# Autodesk Inventor assembly: J005649
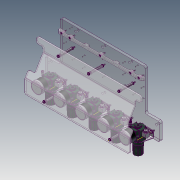
[picture p0: Inventor's stored thumbnail of the model, 180x180]
Saved by Autodesk Inventor 2015 SP1 (Build 190203100, 203)
## iProperties
Created: 2015-05-14
Vendor: HHMI: JRC - ID&F
Document SubType Name: Assembly
Designer: ARNOLDJ
Part Number: J005649
Description: REGULATOR PLATE ASSEMBLY
RuleStatus: InUse
AfterDocSave0: file://Part Number Cleaner
DESIGN DEPARTMENT: HHMI: JRC - ID&F
ALTERED ITEM PART NUMBER: N/A
ALTERED ITEM VENDOR: N/A
ALTERED ITEM DESCRIPTION: N/A
Revision Number: 0
## Documents named in this file (12)
- C:\_WORKSPACE\DATA\COLLABORATION\SVOBODA LAB\MOUSE POSITIONING SYSTEMS\MCAD\BALL SETUP\MBS REG PLATE ASSY.iam
- C:\_WORKSPACE\DATA\COLLABORATION\SVOBODA LAB\MOUSE POSITIONING SYSTEMS\MCAD\BALL SETUP\MBS REG BASE PLATE.ipt
- C:\_WORKSPACE\DATA\COLLABORATION\SVOBODA LAB\MOUSE POSITIONING SYSTEMS\MCAD\BALL SETUP\MBS REGULATOR ASSY.iam
- C:\_WORKSPACE\DATA\COLLABORATION\SVOBODA LAB\MOUSE POSITIONING SYSTEMS\MCAD\BALL SETUP\95947A074.ipt
- C:\_WORKSPACE\DATA\COLLABORATION\SVOBODA LAB\MOUSE POSITIONING SYSTEMS\MCAD\BALL SETUP\93475A230.ipt
- C:\_WORKSPACE\DATA\COLLABORATION\SVOBODA LAB\MOUSE POSITIONING SYSTEMS\MCAD\BALL SETUP\MBS DEFLECTOR SHIELD .ipt
- C:\_WORKSPACE\DATA\COLLABORATION\SVOBODA LAB\MOUSE POSITIONING SYSTEMS\MCAD\BALL SETUP\MBS TROUGH RAIL.ipt
- C:\_WORKSPACE\DATA\COLLABORATION\SVOBODA LAB\MOUSE POSITIONING SYSTEMS\MCAD\BALL SETUP\92010A226.ipt
- C:\_WORKSPACE\DATA\COLLABORATION\SVOBODA LAB\MOUSE POSITIONING SYSTEMS\MCAD\BALL SETUP\92029A152.ipt
- C:\_WORKSPACE\DATA\COLLABORATION\SVOBODA LAB\MOUSE POSITIONING SYSTEMS\MCAD\BALL SETUP\90116A207.ipt
- C:\_WORKSPACE\DATA\COLLABORATION\SVOBODA LAB\MOUSE POSITIONING SYSTEMS\MCAD\BALL SETUP\93475A240.ipt
- C:\_WORKSPACE\DATA\COLLABORATION\SVOBODA LAB\MOUSE POSITIONING SYSTEMS\MCAD\BALL SETUP\92000A320.ipt
## Components (67 placed, 11 different names)
1. MBS REG BASE PLATE:1 — Mate:1, Mate:2, Mate:3, Mate:4, Mate:5, Mate:6, Mate:7, Mate:8, Mate:9, Mate:10, Mate:11, Mate:16, Mate:17, Mate:18, Mate:22, Mate:23, Mate:24, Mate:25, Mate:30, Mate:31, Mate:32, Mate:33, Mate:40, Mate:41, Mate:42, Flush:6, Mate:48, Flush:7, Mate:49, Flush:8, Mate:50, Flush:9, Mate:51, Flush:10, Mate:52
2. 95947A074:1 — Mate:10, Mate:11, Mate:12, Mate:13, Mate:55
3. 95947A074:2 — Mate:12, Mate:13, Mate:19, Mate:20, Mate:21, Mate:54
4. 95947A074:3 — Mate:34, Mate:35, Mate:36, Mate:37, Mate:39
5. 95947A074:4 — Mate:30, Mate:31, Mate:34, Mate:35, Flush:11, Mate:53
6. 95947A074:5 — Mate:4, Mate:5, Mate:28, Mate:29
7. 95947A074:6 — Mate:6, Mate:9, Mate:26, Mate:27
8. 95947A074:7 — Mate:7, Mate:8, Mate:14, Mate:15
9. 93475A230:1 — Mate:14, Mate:15, Mate:65
10. 93475A230:2 — Mate:16, Mate:17
11. 93475A230:3 — Mate:18, Mate:19
12. 93475A230:4 — Mate:28, Mate:29, Mate:63
13. 93475A230:5 — Mate:26, Mate:27, Mate:64
14. 93475A230:6 — Mate:22, Mate:23
15. 93475A230:7 — Mate:24, Mate:25
16. 93475A230:8 — Mate:32, Mate:33
17. 93475A230:9 — Mate:36, Mate:37
18. 93475A230:10 — Mate:20, Mate:21, Mate:38
19. MBS DEFLECTOR SHIELD :1 — Mate:38, Mate:39, Angle:1, Mate:56, Mate:57, Mate:58, Mate:59, Mate:60, Mate:61, Mate:62
20. MBS TROUGH RAIL:1 — Mate:40, Mate:41, Mate:42, Mate:43, Flush:1, Mate:44, Mate:45, Mate:46, Mate:47, Flush:2, Flush:3, Flush:4, Flush:5
21. 92010A226:1 — Mate:43, Flush:1
22. 92010A226:2 — Mate:45, Flush:5
23. 92010A226:3 — Mate:44, Flush:4
24. 92010A226:4 — Mate:46, Flush:3
25. 92010A226:5 — Mate:47, Flush:2
26. 92029A152:1 — Flush:6, Mate:48
27. 92029A152:2 — Flush:7, Mate:49
28. 92029A152:3 — Flush:8, Mate:50
29. 92029A152:4 — Flush:11, Mate:53
30. 92029A152:5 — Mate:54, Mate:55
31. 92029A152:6 — Flush:10, Mate:52
32. 92029A152:9 — Flush:9, Mate:51
33. 93475A230:11 — Mate:57, Mate:63, Mate:70, Mate:71
34. 93475A230:12 — Mate:56, Mate:64, Mate:68, Mate:69
35. 93475A230:13 — Mate:59, Mate:61, Mate:72, Mate:73
36. 93475A230:14 — Mate:58, Mate:65, Mate:66, Mate:67
37. 93475A230:15 — Mate:60, Mate:62, Mate:74, Mate:75
38. 90116A207:1 — Mate:74, Mate:75
39. 90116A207:2 — Mate:72, Mate:73
40. 90116A207:3 — Mate:70, Mate:71
41. 90116A207:4 — Mate:66, Mate:67
42. 90116A207:5 — Mate:68, Mate:69
43. MBS REGULATOR ASSY:1 [sub-assembly] — Mate:1, Mate:2, Mate:3, Mate:76, Mate:77, Mate:78, Mate:79
44. MBS REGULATOR ASSY:2 [sub-assembly]
45. MBS REGULATOR ASSY:3 [sub-assembly]
46. MBS REGULATOR ASSY:4 [sub-assembly]
47. MBS REGULATOR ASSY:5 [sub-assembly]
48. 93475A240:2 — Mate:78, Mate:79, Mate:82, Mate:83
49. 92000A320:2 — Mate:82, Mate:83
50. 93475A240:1 — Mate:76, Mate:77, Mate:80, Mate:81
51. 92000A320:1 — Mate:80, Mate:81
52. 93475A240:3
53. 92000A320:3
54. 93475A240:4
55. 92000A320:4
56. 93475A240:5
57. 92000A320:5
58. 93475A240:6
59. 92000A320:6
60. 93475A240:7
61. 92000A320:7
62. 93475A240:8
63. 92000A320:8
64. 93475A240:9
65. 92000A320:9
66. 93475A240:10
67. 92000A320:10
## Component patterns: (5 elements, first: MBS REGULATOR ASSY:1), (5 elements, first: 93475A240:2 + 92000A320:2 + 93475A240:1 + 92000A320:1)
## Relationships (95: Mate 83, Flush 11, Angle 1)
- Mate:1: MBS REG BASE PLATE:1 ↔ MBS REGULATOR ASSY:1
- Mate:2: MBS REG BASE PLATE:1 ↔ MBS REGULATOR ASSY:1
- Mate:3: MBS REG BASE PLATE:1 ↔ MBS REGULATOR ASSY:1
- Mate:4: MBS REG BASE PLATE:1 ↔ 95947A074:5
- Mate:5 (0.889 mm): MBS REG BASE PLATE:1 ↔ 95947A074:5
- Mate:6: MBS REG BASE PLATE:1 ↔ 95947A074:6
- Mate:7: MBS REG BASE PLATE:1 ↔ 95947A074:7
- Mate:8 (0.889 mm): MBS REG BASE PLATE:1 ↔ 95947A074:7
- Mate:9 (0.889 mm): MBS REG BASE PLATE:1 ↔ 95947A074:6
- Mate:10: MBS REG BASE PLATE:1 ↔ 95947A074:1
- Mate:11 (0.889 mm): MBS REG BASE PLATE:1 ↔ 95947A074:1
- Mate:12: 95947A074:1 ↔ 95947A074:2
- Mate:13: 95947A074:1 ↔ 95947A074:2
- Mate:14: 95947A074:7 ↔ 93475A230:1
- Mate:15: 95947A074:7 ↔ 93475A230:1
- Mate:16: MBS REG BASE PLATE:1 ↔ 93475A230:2
- Mate:17: MBS REG BASE PLATE:1 ↔ 93475A230:2
- Mate:18: MBS REG BASE PLATE:1 ↔ 93475A230:3
- Mate:19: 95947A074:2 ↔ 93475A230:3
- Mate:20: 95947A074:2 ↔ 93475A230:10
- Mate:21: 95947A074:2 ↔ 93475A230:10
- Mate:22: MBS REG BASE PLATE:1 ↔ 93475A230:6
- Mate:23: MBS REG BASE PLATE:1 ↔ 93475A230:6
- Mate:24: MBS REG BASE PLATE:1 ↔ 93475A230:7
- Mate:25: MBS REG BASE PLATE:1 ↔ 93475A230:7
- Mate:26: 95947A074:6 ↔ 93475A230:5
- Mate:27: 95947A074:6 ↔ 93475A230:5
- Mate:28: 95947A074:5 ↔ 93475A230:4
- Mate:29: 95947A074:5 ↔ 93475A230:4
- Mate:30: MBS REG BASE PLATE:1 ↔ 95947A074:4
- Mate:31 (0.889 mm): MBS REG BASE PLATE:1 ↔ 95947A074:4
- Mate:32: MBS REG BASE PLATE:1 ↔ 93475A230:8
- Mate:33: MBS REG BASE PLATE:1 ↔ 93475A230:8
- Mate:34: 95947A074:3 ↔ 95947A074:4
- Mate:35: 95947A074:3 ↔ 95947A074:4
- Mate:36: 95947A074:3 ↔ 93475A230:9
- Mate:37: 95947A074:3 ↔ 93475A230:9
- Mate:38: 93475A230:10 ↔ MBS DEFLECTOR SHIELD :1
- Mate:39: 95947A074:3 ↔ MBS DEFLECTOR SHIELD :1
- Angle:1 (0 deg): MBS DEFLECTOR SHIELD :1
- Mate:40: MBS REG BASE PLATE:1 ↔ MBS TROUGH RAIL:1
- Mate:41: MBS REG BASE PLATE:1 ↔ MBS TROUGH RAIL:1
- Mate:42: MBS REG BASE PLATE:1 ↔ MBS TROUGH RAIL:1
- Mate:43: MBS TROUGH RAIL:1 ↔ 92010A226:1
- Flush:1 (0.889 mm): MBS TROUGH RAIL:1 ↔ 92010A226:1
- Mate:44: MBS TROUGH RAIL:1 ↔ 92010A226:3
- Mate:45: MBS TROUGH RAIL:1 ↔ 92010A226:2
- Mate:46: MBS TROUGH RAIL:1 ↔ 92010A226:4
- Mate:47: MBS TROUGH RAIL:1 ↔ 92010A226:5
- Flush:2 (0.889 mm): MBS TROUGH RAIL:1 ↔ 92010A226:5
- Flush:3 (0.889 mm): MBS TROUGH RAIL:1 ↔ 92010A226:4
- Flush:4 (0.889 mm): MBS TROUGH RAIL:1 ↔ 92010A226:3
- Flush:5 (0.889 mm): MBS TROUGH RAIL:1 ↔ 92010A226:2
- Flush:6 (2.032 mm): MBS REG BASE PLATE:1 ↔ 92029A152:1
- Mate:48: MBS REG BASE PLATE:1 ↔ 92029A152:1
- Flush:7 (2.032 mm): MBS REG BASE PLATE:1 ↔ 92029A152:2
- Mate:49: MBS REG BASE PLATE:1 ↔ 92029A152:2
- Flush:8: MBS REG BASE PLATE:1 ↔ 92029A152:3
- Mate:50: MBS REG BASE PLATE:1 ↔ 92029A152:3
- Flush:9 (2.032 mm): MBS REG BASE PLATE:1 ↔ 92029A152:9
- Mate:51: MBS REG BASE PLATE:1 ↔ 92029A152:9
- Flush:10 (2.032 mm): MBS REG BASE PLATE:1 ↔ 92029A152:6
- Mate:52: MBS REG BASE PLATE:1 ↔ 92029A152:6
- Flush:11 (-8 mm): 95947A074:4 ↔ 92029A152:4
- Mate:53: 95947A074:4 ↔ 92029A152:4
- Mate:54 (-8 mm): 95947A074:2 ↔ 92029A152:5
- Mate:55: 95947A074:1 ↔ 92029A152:5
- Mate:56: MBS DEFLECTOR SHIELD :1 ↔ 93475A230:12
- Mate:57: MBS DEFLECTOR SHIELD :1 ↔ 93475A230:11
- Mate:58: MBS DEFLECTOR SHIELD :1 ↔ 93475A230:14
- Mate:59: MBS DEFLECTOR SHIELD :1 ↔ 93475A230:13
- Mate:60: MBS DEFLECTOR SHIELD :1 ↔ 93475A230:15
- Mate:61: MBS DEFLECTOR SHIELD :1 ↔ 93475A230:13
- Mate:62: MBS DEFLECTOR SHIELD :1 ↔ 93475A230:15
- Mate:63: 93475A230:4 ↔ 93475A230:11
- Mate:64: 93475A230:5 ↔ 93475A230:12
- Mate:65: 93475A230:1 ↔ 93475A230:14
- Mate:66: 93475A230:14 ↔ 90116A207:4
- Mate:67: 93475A230:14 ↔ 90116A207:4
- Mate:68: 93475A230:12 ↔ 90116A207:5
- Mate:69: 93475A230:12 ↔ 90116A207:5
- Mate:70: 93475A230:11 ↔ 90116A207:3
- Mate:71: 93475A230:11 ↔ 90116A207:3
- Mate:72: 93475A230:13 ↔ 90116A207:2
- Mate:73: 93475A230:13 ↔ 90116A207:2
- Mate:74: 93475A230:15 ↔ 90116A207:1
- Mate:75: 93475A230:15 ↔ 90116A207:1
- Mate:76: MBS REGULATOR ASSY:1 ↔ 93475A240:1
- Mate:77: MBS REGULATOR ASSY:1 ↔ 93475A240:1
- Mate:78: MBS REGULATOR ASSY:1 ↔ 93475A240:2
- Mate:79: MBS REGULATOR ASSY:1 ↔ 93475A240:2
- Mate:80: 93475A240:1 ↔ 92000A320:1
- Mate:81: 93475A240:1 ↔ 92000A320:1
- Mate:82: 93475A240:2 ↔ 92000A320:2
- Mate:83: 93475A240:2 ↔ 92000A320:2
